# Autodesk Inventor assembly: zespol_z_lozyskami
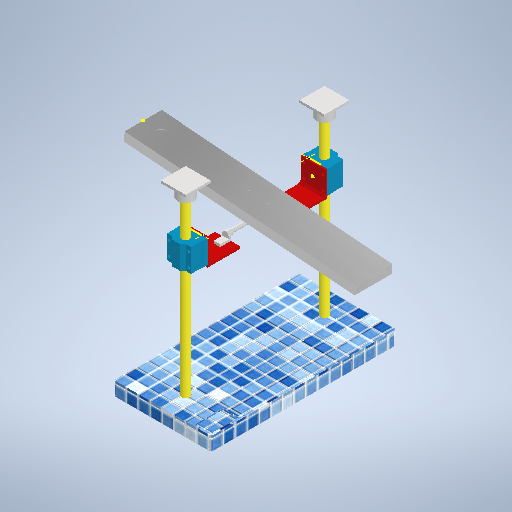
[picture p0: Inventor's stored thumbnail of the model, 512x512]
Saved by Autodesk Inventor 2025 (Build 290162000, 162)
## iProperties
Created: 2024-04-05
Part Number: zespol_z_lozyskami
Document SubType Name: Assembly
Designer: Wojtek
Author: Wojtek
## Documents named in this file (10)
- E:\wazne\inzynierka\kalman-inzynierka\model\zespol_z_lozyskami.iam
- E:\wazne\inzynierka\kalman-inzynierka\model\Podstawa.ipt
- E:\wazne\inzynierka\kalman-inzynierka\model\pret_pionowy.ipt
- E:\wazne\inzynierka\kalman-inzynierka\model\lozysko.ipt
- E:\wazne\inzynierka\kalman-inzynierka\model\obudowa_łoż_pion_1.ipt
- E:\wazne\inzynierka\kalman-inzynierka\model\kapek.ipt
- E:\wazne\inzynierka\kalman-inzynierka\model\chwytak_rurki.ipt
- E:\wazne\inzynierka\kalman-inzynierka\model\kp08\KP08\KP08.iam
- E:\wazne\inzynierka\kalman-inzynierka\model\pret_krotki.ipt
- E:\wazne\inzynierka\kalman-inzynierka\model\belka.ipt
## Components (14 placed, 9 different names)
1. Podstawa:1 — Wstawiające:1, Wstawiające:2
2. pret_pionowy:1 — Wstawiające:2, Wstawiające:4, Wstawiające:11
3. pret_pionowy:2 — Wstawiające:1, Wstawiające:3, Równoległe:1, Wstawiające:10
4. lozysko:1 — Wstawiające:3, Równoległe:1, Wstawiające:5, Wstawiające:9
5. lozysko:2 — Wstawiające:4, Wstawiające:7, Wstawiające:8
6. obudowa_łoż_pion_1:1 — Wstawiające:7, Wstawiające:8, Zestawiające:3, Zestawiające:4, Równoległe:3, Równoległe:4
7. obudowa_łoż_pion_1:2 — Wstawiające:5, Wstawiające:9, Zestawiające:1, Zestawiające:2, Równoległe:2, Równoległe:4
8. kapek:1 — Wstawiające:10
9. kapek:2 — Wstawiające:11
10. chwytak_rurki:1 — Zestawiające:1, Zestawiające:2, Równoległe:2
11. chwytak_rurki:2 — Zestawiające:3, Zestawiające:4, Równoległe:3, Wstawiające:13
12. KP08:1 [sub-assembly] — Wstawiające:12, Wstawiające:14
13. pret_krotki:1 — Wstawiające:12, Wstawiające:13
14. belka:1 — Wstawiające:14
## Relationships (21: Insert 13, Flush 4, Mate 4)
- Wstawiające:1 [Insert]: Podstawa:1 ↔ pret_pionowy:2
- Wstawiające:2 [Insert]: Podstawa:1 ↔ pret_pionowy:1
- Wstawiające:3 [Insert] (100 mm): pret_pionowy:2 ↔ lozysko:1
- Wstawiające:4 [Insert] (100 mm): pret_pionowy:1 ↔ lozysko:2
- Równoległe:1 [Flush]: pret_pionowy:2 ↔ lozysko:1
- Wstawiające:5 [Insert] (-2 mm): lozysko:1 ↔ obudowa_łoż_pion_1:2
- Wstawiające:7 [Insert] (-2 mm): lozysko:2 ↔ obudowa_łoż_pion_1:1
- Wstawiające:8 [Insert] (-2 mm): lozysko:2 ↔ obudowa_łoż_pion_1:1
- Wstawiające:9 [Insert] (-2 mm): lozysko:1 ↔ obudowa_łoż_pion_1:2
- Wstawiające:10 [Insert] (-25 mm): pret_pionowy:2 ↔ kapek:1
- Wstawiające:11 [Insert] (-25 mm): pret_pionowy:1 ↔ kapek:2
- Zestawiające:1 [Mate]: obudowa_łoż_pion_1:2 ↔ chwytak_rurki:1
- Zestawiające:2 [Mate] (45 mm): obudowa_łoż_pion_1:2 ↔ chwytak_rurki:1
- Równoległe:2 [Flush] (20 mm): obudowa_łoż_pion_1:2 ↔ chwytak_rurki:1
- Zestawiające:3 [Mate] (45 mm): obudowa_łoż_pion_1:1 ↔ chwytak_rurki:2
- Zestawiające:4 [Mate]: obudowa_łoż_pion_1:1 ↔ chwytak_rurki:2
- Równoległe:3 [Flush] (20 mm): obudowa_łoż_pion_1:1 ↔ chwytak_rurki:2
- Wstawiające:12 [Insert] (-60 mm): KP08:1 ↔ pret_krotki:1
- Wstawiające:13 [Insert] (-5 mm): chwytak_rurki:2 ↔ pret_krotki:1
- Równoległe:4 [Flush]: obudowa_łoż_pion_1:1 ↔ obudowa_łoż_pion_1:2
- Wstawiające:14 [Insert]: KP08:1 ↔ belka:1
